# Autodesk Inventor assembly: idler
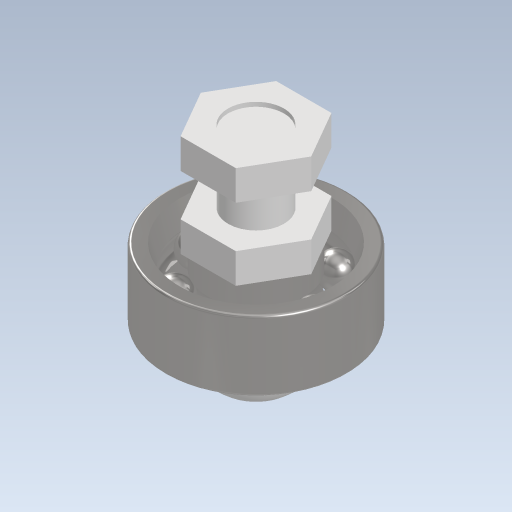
[picture p0: Inventor's stored thumbnail of the model, 512x512]
Saved by Autodesk Inventor 2023 (Build 270158000, 158)
## iProperties
Created: 2023-05-19
Part Number: idler
Document SubType Name: Assembly
Designer: Johnny Jou
Author: Johnny Jou
## Documents named in this file (4)
- C:\Users\Johnny Jou\Documents\GitHub\Areo_Rider_Cabin\Expansion\test\idler.iam
- C:\Users\Johnny Jou\Documents\GitHub\Areo_Rider_Cabin\Expansion\test\screw_4_12.ipt
- C:\Users\Johnny Jou\Documents\GitHub\Areo_Rider_Cabin\car\bearing.ipt
- C:\Users\Johnny Jou\Documents\GitHub\Areo_Rider_Cabin\Expansion\test\nut_thin_M4.ipt
## Components (4 placed, 3 different names)
1. screw_4_12:1
2. 軸承 GB/T 292-2007 類型 IN - 退回 B724 C:1
3. nut_thin_M4:1
4. nut_thin_M4:2
## Relationships (4: Insert 2, Mate 2)
- [Insert]: screw_4_12:1 ↔ 軸承 GB/T 292-2007 類型 IN - 退回 B724 C:1
- [Insert]: 軸承 GB/T 292-2007 類型 IN - 退回 B724 C:1 ↔ nut_thin_M4:1
- [Mate]: screw_4_12:1 ↔ nut_thin_M4:2
- [Mate] (3 mm): nut_thin_M4:1 ↔ nut_thin_M4:2
